# Autodesk Inventor assembly: carrom_bot 1
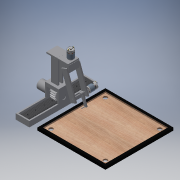
[picture p0: Inventor's stored thumbnail of the model, 180x180]
Saved by Autodesk Inventor 2019.4 (Build 234330000, 330)
## iProperties
Created: 2020-04-16
Part Number: carrom_bot 1
Document SubType Name: Assembly
Designer: Niran
Author: Niran
## iProperties of the stored document S.Carrom board.ipt
Created: 2015-04-24
Part Number: S.Carrom board
Material: Birch
Document SubType Name: Modeling
Designer: sandeep suddarsi
Density: 0.512 g/cm^3
Appearance: Default
Author: sandeep suddarsi
Sending System: Autodesk Inventor 2020
## Documents named in this file (4)
- **C:\Users\Niran\Desktop\S.Carrom_bot\carrom_bot 1.iam*LocalDocs*x3vc1hjfwKiqyeysoJutwkl0bUb*S.Carrom board.ipt
- C:\Users\Niran\Desktop\S.Carrom_bot\carrom_bot 1.iam
- C:\Users\Niran\Desktop\S.Carrom_bot\carrom_bot.iam
- C:\Users\Niran\Desktop\S.Carrom_bot\S.Carrom board.ipt
## Components (2 placed, 2 different names)
1. carrom_bot:1 [sub-assembly] — Rigid:1
2. S.Carrom board:1 — Rigid:1
## Relationships (1: WeldJoint 1)
- Rigid:1 [WeldJoint] (60 mm): carrom_bot:1 ↔ S.Carrom board:1
